# Autodesk Inventor assembly: 000-install-encoder-v1
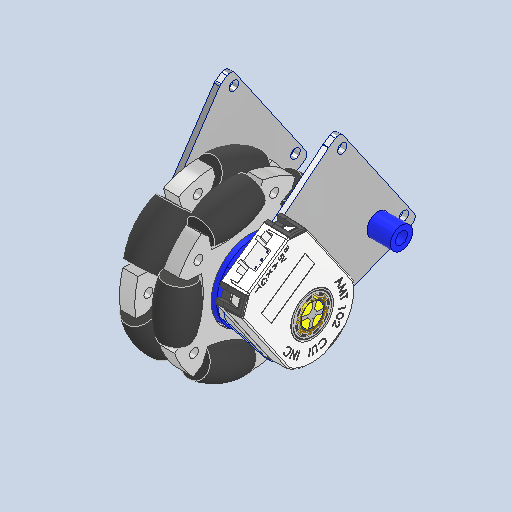
[picture p0: Inventor's stored thumbnail of the model, 512x512]
Saved by Autodesk Inventor 2025.2 (Build 292293000, 293)
## iProperties
Created: 2024-02-12
Part Number: 000-install-encoder-v1
Document SubType Name: Assembly
Designer: haruy
Author: haruy
## Documents named in this file (9)
- C:\Users\haruy\Documents\ロボコン\NHK2025\cad\nagahisa\odom\000-install-encoder-v1.iam
- C:\Users\haruy\Documents\ロボコン\NHK2025\cad\nagahisa\odom\install-encoder-v1-3DP-Shaft-F.ipt
- C:\Users\haruy\Documents\ロボコン\NHK2025\cad\nagahisa\odom\omni-60.ipt
- C:\Users\haruy\Documents\ロボコン\NHK2025\cad\nagahisa\odom\install-encoder-v1-Plate-E-F.ipt
- C:\Users\haruy\Documents\ロボコン\NHK2025\cad\nagahisa\odom\install-encoder-v1-Plate-E-F-R.ipt
- C:\Users\haruy\Documents\ロボコン\NHK2025\cad\nagahisa\odom\install-encoder-v1-Shaft-E-Shaft.ipt
- C:\Users\haruy\Documents\ロボコン\NHK2025\cad\nagahisa\odom\bear_f8_12_sa.ipt
- C:\Users\haruy\Documents\ロボコン\NHK2025\cad\nagahisa\odom\amt102-v.iam
- C:\Users\haruy\Documents\ロボコン\NHK2025\cad\nagahisa\odom\install-encoder-v1-3DP-Spacer-down.ipt
## Components (9 placed, 8 different names)
1. install-encoder-v1-3DP-Shaft-F:1 — 挿入:1, 挿入:2, 挿入:7
2. omni-60:1 — 挿入:1, 挿入:2
3. install-encoder-v1-Plate-E-F:1 — 挿入:4, 挿入:10, 挿入:14
4. install-encoder-v1-Plate-E-F-R:1 — 挿入:3
5. install-encoder-v1-Shaft-E-Shaft:1 — 挿入:5, 挿入:6, 挿入:7
6. bear_f8_12_sa:1 — 挿入:4, 挿入:6
7. bear_f8_12_sa:2 — 挿入:3, 挿入:5
8. amt102-v:1 [sub-assembly] — 挿入:10
9. install-encoder-v1-3DP-Spacer-down:1 — 挿入:14
## Relationships (9: Insert 9)
- 挿入:1 [Insert]: install-encoder-v1-3DP-Shaft-F:1 ↔ omni-60:1
- 挿入:2 [Insert]: install-encoder-v1-3DP-Shaft-F:1 ↔ omni-60:1
- 挿入:3 [Insert]: install-encoder-v1-Plate-E-F-R:1 ↔ bear_f8_12_sa:2
- 挿入:4 [Insert]: install-encoder-v1-Plate-E-F:1 ↔ bear_f8_12_sa:1
- 挿入:5 [Insert]: install-encoder-v1-Shaft-E-Shaft:1 ↔ bear_f8_12_sa:2
- 挿入:6 [Insert]: install-encoder-v1-Shaft-E-Shaft:1 ↔ bear_f8_12_sa:1
- 挿入:7 [Insert] (3 mm): install-encoder-v1-3DP-Shaft-F:1 ↔ install-encoder-v1-Shaft-E-Shaft:1
- 挿入:10 [Insert]: install-encoder-v1-Plate-E-F:1 ↔ amt102-v:1
- 挿入:14 [Insert]: install-encoder-v1-Plate-E-F:1 ↔ install-encoder-v1-3DP-Spacer-down:1
